# Autodesk Inventor assembly: X02598_LEGOmini_LowerBody
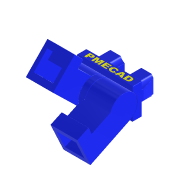
[picture p0: Inventor's stored thumbnail of the model, 180x180]
Saved by Autodesk Inventor 2022.2 (Build 262287000, 287)
## iProperties
Created: 2022-02-05
Part Number: X02598_LEGOmini_LowerBody
Document SubType Name: Assembly
Designer: Jason
Author: Jason
## Documents named in this file (4)
- C:\Users\Jason\Documents\PME1017_X02598\教材_LEGOmini_20220205\X02598_LEGOmini_LowerBody.iam
- C:\Users\Jason\Documents\PME1017_X02598\教材_LEGOmini_20220205\X02598_LEGOmini_Waist_B.ipt
- C:\Users\Jason\Documents\PME1017_X02598\教材_LEGOmini_20220205\X02598_LEGOmini_RightLeg_B.ipt
- C:\Users\Jason\Documents\PME1017_X02598\教材_LEGOmini_20220205\X02598_LEGOmini_LeftLeg_B.ipt
## Components (3 placed, 3 different names)
1. X02598_LEGOmini_Waist_B:1 — 插入:1, 插入:2
2. X02598_LEGOmini_RightLeg_B:1 — 插入:1
3. X02598_LEGOmini_LeftLeg_B:1 — 插入:2
## Relationships (2: Insert 2)
- 插入:1 [Insert]: X02598_LEGOmini_Waist_B:1 ↔ X02598_LEGOmini_RightLeg_B:1
- 插入:2 [Insert]: X02598_LEGOmini_Waist_B:1 ↔ X02598_LEGOmini_LeftLeg_B:1
